# Autodesk Inventor assembly: 211-01
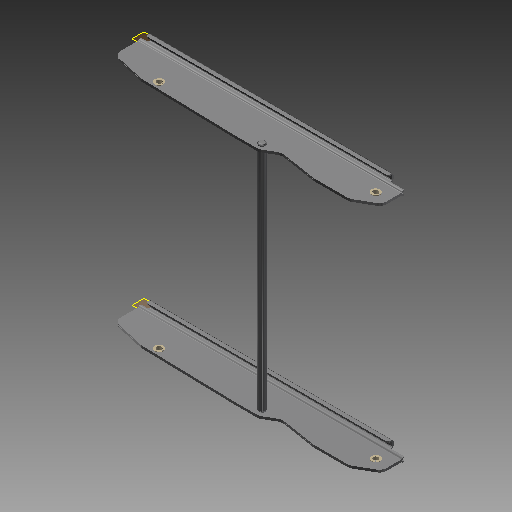
[picture p0: Inventor's stored thumbnail of the model, 512x512]
Saved by Autodesk Inventor 2019 (Build 230136000, 136)
## iProperties
Company: Autodesk Inc.
Created: 2007-12-24
Part Number: 211-01
Document SubType Name: Assembly
Designer: Autodesk Inc.
Mass: 2391.73 g
Surface Area: 2865.33 cm^2
Volume: 304.601 cm^3
Density: 7.85201 g/cm^3
Description: BOTTOM GUIDE RAIL ASSEMBLY
Component Category: Lower Component
Author: Inventor
## Documents named in this file (5)
- C:\TEMP\Car Seat\Workspace\Bottom Guide Rail Assembly.iam
- C:\TEMP\Car Seat\Workspace\Chassis Base R.ipt
- C:\TEMP\Car Seat\Workspace\Chassis Base L.ipt
- C:\TEMP\Car Seat\Workspace\Support Rod.ipt
- C:\TEMP\Car Seat\Workspace\Bushing 1.ipt
## Components (9 placed, 4 different names)
1. Chassis Base R:1 — Insert:6, Insert:7, Insert:8, Mate:5, Flush:6, Mate:8
2. Support Rod:1 — Insert:6, Insert:10, Flush:7
3. Bushing 1:1 — Insert:7, Mate:6
4. Bushing 1:2 — Insert:8, Insert:9
5. Bushing 1:3 — Insert:12, Insert:13
6. Bushing 1:4 — Insert:11, Mate:7
7. Chassis Base L:1 — Insert:9, Mate:6
8. Chassis Base R:2 — Insert:13, Mate:7
9. Chassis Base L:2 — Insert:10, Flush:6, Insert:11, Insert:12
## Relationships (14: Insert 8, Mate 4, Flush 2)
- Insert:6: Chassis Base R:1 ↔ Support Rod:1
- Insert:7: Chassis Base R:1 ↔ Bushing 1:1
- Insert:8: Chassis Base R:1 ↔ Bushing 1:2
- Insert:9: Bushing 1:2 ↔ Chassis Base L:1
- Mate:5: Chassis Base R:1
- Mate:6: Bushing 1:1 ↔ Chassis Base L:1
- Insert:10: Support Rod:1 ↔ Chassis Base L:2
- Flush:6: Chassis Base R:1 ↔ Chassis Base L:2
- Insert:11: Bushing 1:4 ↔ Chassis Base L:2
- Insert:12: Bushing 1:3 ↔ Chassis Base L:2
- Insert:13: Bushing 1:3 ↔ Chassis Base R:2
- Mate:7: Bushing 1:4 ↔ Chassis Base R:2
- Mate:8: Chassis Base R:1
- Flush:7: Support Rod:1
